# Autodesk Inventor assembly: Gearbox
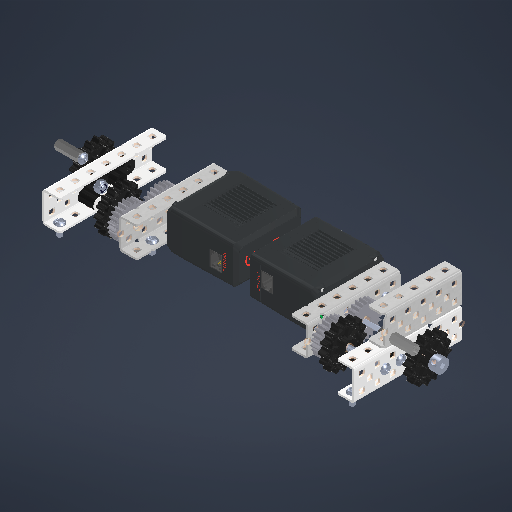
[picture p0: Inventor's stored thumbnail of the model, 512x512]
Saved by Autodesk Inventor 2025 (Build 290162000, 162)
## iProperties
Created: 2024-12-19
Part Number: Gearbox
Document SubType Name: Assembly
Designer: Juan
Author: Juan
## Documents named in this file (34)
- C:\Users\Juan\Documents\GitHub\ATUM-VRC-High-Stakes-CAD\Protobot\Gearbox.iam
- C:\Users\Juan\Documents\GitHub\ATUM-VRC-High-Stakes-CAD\VEX-CAD-Inventor\Motion\Sprockets\6P Sprocket\6P 16T Sprocket, No Insert.iam
- C:\Users\Juan\Documents\GitHub\ATUM-VRC-High-Stakes-CAD\VEX-CAD-Inventor\Motion\Sprockets\6P Sprocket.iam
- C:\Users\Juan\Documents\GitHub\ATUM-VRC-High-Stakes-CAD\VEX-CAD-Inventor\Electronics\Motors with Screws\SteelM-StarS.iam
- C:\Users\Juan\Documents\GitHub\ATUM-VRC-High-Stakes-CAD\VEX-CAD-Inventor\Electronics\Motors with Screws.iam
- C:\Users\Juan\Documents\GitHub\ATUM-VRC-High-Stakes-CAD\VEX-CAD-Inventor\Structure\C Channel\Aluminum 1x2x1\Alu C 1x2x1x6.ipt
- C:\Users\Juan\Documents\GitHub\ATUM-VRC-High-Stakes-CAD\Protobot\Half Cut 24t.iam
- C:\Users\Juan\Documents\GitHub\ATUM-VRC-High-Stakes-CAD\VEX-CAD-Inventor\Motion\Insert Circle.ipt
- C:\Users\Juan\Documents\GitHub\ATUM-VRC-High-Stakes-CAD\VEX-CAD-Inventor\Structure\C Channel\Aluminum 1x2x1\Alu C 1x2x1x7.ipt
- C:\Users\Juan\Documents\GitHub\ATUM-VRC-High-Stakes-CAD\VEX-CAD-Inventor\Motion\Spacers\Spacer Nylon .375 OD\NSpacer .375 OD x .125.ipt
- C:\Users\Juan\Documents\GitHub\ATUM-VRC-High-Stakes-CAD\VEX-CAD-Inventor\Motion\Spacers\Spacer Nylon .375 OD.ipt
- C:\Users\Juan\Documents\GitHub\ATUM-VRC-High-Stakes-CAD\VEX-CAD-Inventor\Motion\Spacers\Washer Teflon\TWasher .375 OD x .06250.ipt
- C:\Users\Juan\Documents\GitHub\ATUM-VRC-High-Stakes-CAD\VEX-CAD-Inventor\Motion\Spacers\Washer Teflon.ipt
- C:\Users\Juan\Documents\GitHub\ATUM-VRC-High-Stakes-CAD\VEX-CAD-Inventor\Motion\Spacers\Washer Steel\SWasher .375 OD x .062500.ipt
- C:\Users\Juan\Documents\GitHub\ATUM-VRC-High-Stakes-CAD\VEX-CAD-Inventor\Motion\Spacers\Washer Steel.ipt
- C:\Users\Juan\Documents\GitHub\ATUM-VRC-High-Stakes-CAD\VEX-CAD-Inventor\Motion\Shaft LS\Bearing Flat.ipt
- C:\Users\Juan\Documents\GitHub\ATUM-VRC-High-Stakes-CAD\VEX-CAD-Inventor\Structure\Hardware\Screw Steel - Star\SScrew Star Threaded .500.ipt
- C:\Users\Juan\Documents\GitHub\ATUM-VRC-High-Stakes-CAD\VEX-CAD-Inventor\Structure\Hardware\Screw Steel - Star.ipt
- C:\Users\Juan\Documents\GitHub\ATUM-VRC-High-Stakes-CAD\VEX-CAD-Inventor\Structure\Hardware\Nut Thin Nylock.ipt
- C:\Users\Juan\Documents\GitHub\ATUM-VRC-High-Stakes-CAD\VEX-CAD-Inventor\Structure\Hardware\Screw Steel - Star\SScrew Star Threaded 2.250.ipt
- C:\Users\Juan\Documents\GitHub\ATUM-VRC-High-Stakes-CAD\VEX-CAD-Inventor\Structure\Hardware\Nut Nylock.ipt
- C:\Users\Juan\Documents\GitHub\ATUM-VRC-High-Stakes-CAD\VEX-CAD-Inventor\Motion\Spacers\Spacer Nylon .375 OD\NSpacer .375 OD x .500.ipt
- C:\Users\Juan\Documents\GitHub\ATUM-VRC-High-Stakes-CAD\VEX-CAD-Inventor\Motion\Spacers\Washer Teflon\TWasher .375 OD x .03125.ipt
- C:\Users\Juan\Documents\GitHub\ATUM-VRC-High-Stakes-CAD\VEX-CAD-Inventor\Motion\Shaft LS\Shaft LS\Shaft LS 3.5.ipt
- C:\Users\Juan\Documents\GitHub\ATUM-VRC-High-Stakes-CAD\VEX-CAD-Inventor\Motion\Shaft LS\Shaft LS.ipt
- C:\Users\Juan\Documents\GitHub\ATUM-VRC-High-Stakes-CAD\VEX-CAD-Inventor\Motion\Spacers\Spacer Nylon .375 OD\NSpacer .375 OD x .250.ipt
- C:\Users\Juan\Documents\GitHub\ATUM-VRC-High-Stakes-CAD\VEX-CAD-Inventor\Motion\Sprockets\6P Sprocket\6P 8T Sprocket, Square.iam
- C:\Users\Juan\Documents\GitHub\ATUM-VRC-High-Stakes-CAD\VEX-CAD-Inventor\Motion\Spacers\Spacer Nylon .500 OD\NSpacer Black .500 OD x .125.ipt
- C:\Users\Juan\Documents\GitHub\ATUM-VRC-High-Stakes-CAD\VEX-CAD-Inventor\Motion\Spacers\Spacer Nylon .500 OD.ipt
- C:\Users\Juan\Documents\GitHub\ATUM-VRC-High-Stakes-CAD\VEX-CAD-Inventor\Structure\C Channel\Aluminum 1x2x1\Alu C 1x2x1x5.ipt
- C:\Users\Juan\Documents\GitHub\ATUM-VRC-High-Stakes-CAD\VEX-CAD-Inventor\Structure\Standoff\Standoff .75.ipt
- C:\Users\Juan\Documents\GitHub\ATUM-VRC-High-Stakes-CAD\VEX-CAD-Inventor\Structure\Standoff.ipt
- C:\Users\Juan\Documents\GitHub\ATUM-VRC-High-Stakes-CAD\VEX-CAD-Inventor\Motion\Shaft LS\Shaft Collar Metal\Shaft Collar No Screw.ipt
- C:\Users\Juan\Documents\GitHub\ATUM-VRC-High-Stakes-CAD\VEX-CAD-Inventor\Structure\Hardware\Screw Steel - Star\SScrew Star Smooth .375.ipt
## Components (51 placed, 24 different names)
1. 6P 16T Sprocket, No Insert:1 [sub-assembly]
2. SteelM-StarS:1 [sub-assembly]
3. Alu C 1x2x1x6:1
4. Half Cut 24t:1 [sub-assembly]
5. Half Cut 24t:2 [sub-assembly]
6. Insert Circle:1
7. Alu C 1x2x1x7:1
8. NSpacer .375 OD x .125:1
9. TWasher .375 OD x .06250:1
10. SWasher .375 OD x .062500:1
11. SWasher .375 OD x .062500:2
12. Bearing Flat:1
13. SScrew Star Threaded .500:1
14. Nut Thin Nylock:1
15. SScrew Star Threaded 2.250:2
16. Nut Nylock:1
17. NSpacer .375 OD x .500:2
18. TWasher .375 OD x .03125:2
19. Shaft LS 3.5:1
20. Half Cut 24t:3 [sub-assembly]
21. 6P 16T Sprocket, No Insert:2 [sub-assembly]
22. SteelM-StarS:2 [sub-assembly]
23. Alu C 1x2x1x6:2
24. Insert Circle:2
25. Alu C 1x2x1x7:2
26. TWasher .375 OD x .06250:3
27. SWasher .375 OD x .062500:3
28. SWasher .375 OD x .062500:4
29. SScrew Star Threaded .500:3
30. NSpacer .375 OD x .500:3
31. TWasher .375 OD x .03125:4
32. Bearing Flat:2
33. Half Cut 24t:4 [sub-assembly]
34. Nut Thin Nylock:2
35. NSpacer .375 OD x .250:4
36. NSpacer .375 OD x .250:5
37. 6P 8T Sprocket, Square:3 [sub-assembly]
38. 6P 16T Sprocket, No Insert:4 [sub-assembly]
39. NSpacer Black .500 OD x .125:1
40. 6P 16T Sprocket, No Insert:5 [sub-assembly]
41. NSpacer Black .500 OD x .125:2
42. Alu C 1x2x1x5:1
43. Standoff .75:1
44. Standoff .75:2
45. Shaft Collar No Screw:1
46. SScrew Star Smooth .375:4
47. SScrew Star Smooth .375:5
48. SScrew Star Smooth .375:6
49. SScrew Star Smooth .375:7
50. SScrew Star Smooth .375:8
51. SScrew Star Smooth .375:9
## Relationships (80: Mate 74, WeldJoint 4, Flush 1, Angle 1)
- [Mate]: SteelM-StarS:1 ↔ Alu C 1x2x1x6:1
- [Mate]: SteelM-StarS:1 ↔ Alu C 1x2x1x6:1
- [Mate]: Half Cut 24t:2 ↔ Insert Circle:1
- [Mate]: Half Cut 24t:2 ↔ Insert Circle:1
- [Mate]: 6P 16T Sprocket, No Insert:1 ↔ Half Cut 24t:2
- [Mate]: Alu C 1x2x1x6:1 ↔ Half Cut 24t:1
- [Mate]: Alu C 1x2x1x6:1 ↔ Alu C 1x2x1x7:1
- [Mate]: Alu C 1x2x1x6:1 ↔ Alu C 1x2x1x7:1
- [Mate]: Half Cut 24t:1 ↔ NSpacer .375 OD x .125:1
- [Mate]: Alu C 1x2x1x6:1 ↔ NSpacer .375 OD x .125:1
- [Mate]: Half Cut 24t:1 ↔ NSpacer .375 OD x .125:1
- [Mate]: Alu C 1x2x1x6:1 ↔ TWasher .375 OD x .06250:1
- [Mate]: Insert Circle:1 ↔ TWasher .375 OD x .06250:1
- [Mate]: Alu C 1x2x1x6:1 ↔ SWasher .375 OD x .062500:1
- [Mate]: Alu C 1x2x1x6:1 ↔ SWasher .375 OD x .062500:2
- [Mate]: Alu C 1x2x1x7:1 ↔ Bearing Flat:1
- [Mate]: Alu C 1x2x1x7:1 ↔ Bearing Flat:1
- [Mate]: Alu C 1x2x1x7:1 ↔ Bearing Flat:1
- [Mate]: Alu C 1x2x1x7:1 ↔ SScrew Star Threaded .500:1
- [Mate]: Alu C 1x2x1x7:1 ↔ SScrew Star Threaded .500:1
- [Mate]: SScrew Star Threaded .500:1 ↔ Nut Thin Nylock:1
- [Mate]: Bearing Flat:1 ↔ Nut Thin Nylock:1
- [Mate]: Alu C 1x2x1x7:1 ↔ SScrew Star Threaded 2.250:2
- [Mate]: Alu C 1x2x1x7:1 ↔ SScrew Star Threaded 2.250:2
- [Mate]: SScrew Star Threaded 2.250:2 ↔ Nut Nylock:1
- [Mate]: Alu C 1x2x1x7:1 ↔ Nut Nylock:1
- [Mate]: SScrew Star Threaded 2.250:2 ↔ NSpacer .375 OD x .500:2
- [Mate]: Nut Nylock:1 ↔ NSpacer .375 OD x .500:2
- [Mate]: NSpacer .375 OD x .500:2 ↔ TWasher .375 OD x .03125:2
- [Mate]: NSpacer .375 OD x .500:2 ↔ TWasher .375 OD x .03125:2
- [Mate]: Half Cut 24t:1 ↔ Shaft LS 3.5:1
- [Flush]: Shaft LS 3.5:1 ↔ Shaft Collar No Screw:1
- [Mate]: Alu C 1x2x1x6:1 ↔ Insert Circle:1
- [Mate]: SteelM-StarS:2 ↔ Alu C 1x2x1x6:2
- [Mate]: SteelM-StarS:2 ↔ Alu C 1x2x1x6:2
- [Mate]: Half Cut 24t:3 ↔ Alu C 1x2x1x6:2
- [Mate]: Alu C 1x2x1x6:2 ↔ Insert Circle:2
- [Mate]: Alu C 1x2x1x6:2 ↔ Alu C 1x2x1x7:2
- [Mate]: Alu C 1x2x1x6:2 ↔ Alu C 1x2x1x7:2
- [Mate]: Insert Circle:2 ↔ TWasher .375 OD x .06250:3
- [Mate]: Alu C 1x2x1x6:2 ↔ TWasher .375 OD x .06250:3
- [Mate]: Alu C 1x2x1x6:2 ↔ SWasher .375 OD x .062500:3
- [Mate]: Alu C 1x2x1x6:2 ↔ SWasher .375 OD x .062500:4
- [Mate]: Alu C 1x2x1x7:2 ↔ SScrew Star Threaded .500:3
- [Mate]: Alu C 1x2x1x7:2 ↔ SScrew Star Threaded .500:3
- [Mate]: NSpacer .375 OD x .500:3 ↔ TWasher .375 OD x .03125:4
- [Mate]: NSpacer .375 OD x .500:3 ↔ TWasher .375 OD x .03125:4
- [Mate]: Alu C 1x2x1x7:2 ↔ Bearing Flat:2
- [Mate]: Alu C 1x2x1x7:2 ↔ Bearing Flat:2
- [Mate]: Alu C 1x2x1x6:2 ↔ SWasher .375 OD x .062500:3
- [Mate]: SteelM-StarS:2 ↔ Alu C 1x2x1x6:2
- [Mate]: Insert Circle:2 ↔ Half Cut 24t:4
- [Mate]: Alu C 1x2x1x6:2 ↔ TWasher .375 OD x .06250:3
- [Mate]: TWasher .375 OD x .06250:3 ↔ Half Cut 24t:4
- [Mate]: 6P 16T Sprocket, No Insert:2 ↔ Half Cut 24t:4
- [Mate]: Bearing Flat:2 ↔ Nut Thin Nylock:2
- [Mate]: SScrew Star Threaded .500:3 ↔ Nut Thin Nylock:2
- [Mate]: Alu C 1x2x1x7:2 ↔ Bearing Flat:2
- [Mate]: Bearing Flat:1 ↔ NSpacer .375 OD x .250:4
- [Mate]: Bearing Flat:1 ↔ NSpacer .375 OD x .250:4
- [Mate]: Bearing Flat:2 ↔ NSpacer .375 OD x .250:5
- [Mate]: Bearing Flat:2 ↔ NSpacer .375 OD x .250:5
- [Mate]: Alu C 1x2x1x7:1 ↔ 6P 8T Sprocket, Square:3
- [Mate]: NSpacer .375 OD x .250:4 ↔ 6P 8T Sprocket, Square:3
- [Mate]: Alu C 1x2x1x7:1 ↔ 6P 16T Sprocket, No Insert:4
- [Mate]: Alu C 1x2x1x7:1 ↔ NSpacer Black .500 OD x .125:1
- [Mate]: Alu C 1x2x1x7:1 ↔ NSpacer Black .500 OD x .125:1
- [Mate]: Alu C 1x2x1x7:2 ↔ 6P 16T Sprocket, No Insert:5
- [Mate]: Alu C 1x2x1x7:2 ↔ NSpacer Black .500 OD x .125:2
- [Mate]: 6P 16T Sprocket, No Insert:5 ↔ NSpacer Black .500 OD x .125:2
- [Mate]: Alu C 1x2x1x7:1 ↔ Alu C 1x2x1x5:1
- [Mate]: Alu C 1x2x1x7:1 ↔ Alu C 1x2x1x5:1
- [Mate]: Alu C 1x2x1x7:1 ↔ Alu C 1x2x1x5:1
- [Mate]: Alu C 1x2x1x5:1 ↔ Standoff .75:1
- [Mate]: Alu C 1x2x1x5:1 ↔ Standoff .75:1
- [WeldJoint]: 6P 16T Sprocket, No Insert:4 ↔ Shaft Collar No Screw:1
- [WeldJoint]: Alu C 1x2x1x5:1 ↔ SScrew Star Smooth .375:5
- [WeldJoint]: Alu C 1x2x1x7:1 ↔ SScrew Star Smooth .375:7
- [WeldJoint]: Alu C 1x2x1x6:1 ↔ SScrew Star Smooth .375:6
- [Angle] (0 deg): Shaft LS 3.5:1 ↔ Shaft Collar No Screw:1
